# Autodesk Inventor assembly: claws_endeffector_4
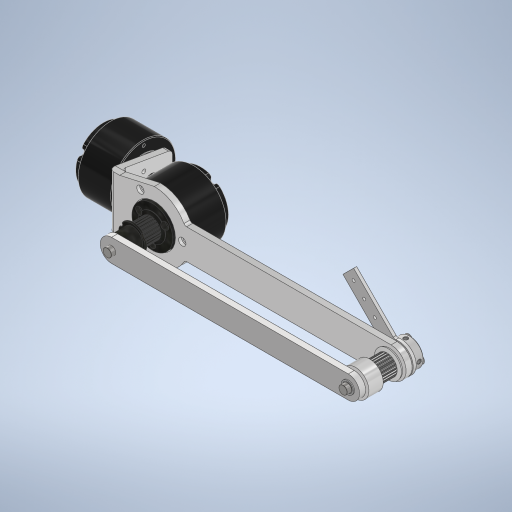
[picture p0: Inventor's stored thumbnail of the model, 512x512]
Saved by Autodesk Inventor 2024 (Build 280153000, 153)
## iProperties
Created: 2025-03-25
Part Number: claws_endeffector_4
Document SubType Name: Assembly
Designer: 1412z
Author: 1412z
## Documents named in this file (13)
- C:\Users\1412z\OneDrive\デスクトップ\rdclab\harvesting_robot\harvesting_endeffector\claws_endeffector\claws_endeffector_4.iam
- C:\Users\1412z\OneDrive\デスクトップ\rdclab\harvesting_robot\harvesting_endeffector\claws_endeffector\motor_holder\motor_holder_4.ipt
- C:\Users\1412z\OneDrive\デスクトップ\rdclab\harvesting_robot\harvesting_endeffector\claws_endeffector\GIM3505-08\GIM3505-8_with-driver.ipt
- C:\Users\1412z\OneDrive\デスクトップ\rdclab\harvesting_robot\harvesting_endeffector\claws_endeffector\misumi\SFL674ZZ_Autodesk_Inventor_2024_20250304\SFL674ZZ.ipt
- C:\Users\1412z\OneDrive\デスクトップ\rdclab\harvesting_robot\harvesting_endeffector\claws_endeffector\misumi\simring\simring_Φ4-Φ5.ipt
- C:\Users\1412z\OneDrive\デスクトップ\rdclab\harvesting_robot\harvesting_endeffector\claws_endeffector\misumi\HTPA22S2M100-K-P4_Autodesk_Inventor_2024_20250304\AIS2024\HTPA22S2M100-K-P4_a.ipt
- C:\Users\1412z\OneDrive\デスクトップ\rdclab\harvesting_robot\harvesting_endeffector\claws_endeffector\cutter_part\cutter_board.ipt
- C:\Users\1412z\OneDrive\デスクトップ\rdclab\harvesting_robot\harvesting_endeffector\claws_endeffector\misumi\SSCMN4_Autodesk_Inventor_2024_20250310\AIS2024\SSCMN4b.ipt
- C:\Users\1412z\OneDrive\デスクトップ\rdclab\harvesting_robot\harvesting_endeffector\claws_endeffector\misumi\M3×8\M3×8.ipt
- C:\Users\1412z\OneDrive\デスクトップ\rdclab\harvesting_robot\harvesting_endeffector\claws_endeffector\misumi\HTPA22S2M100-A-V4-Z6-J3_Autodesk_Inventor_2024_20250304\HTPA22S2M100-A-V4-Z6-J3_0_a-2.ipt
- C:\Users\1412z\OneDrive\デスクトップ\rdclab\harvesting_robot\harvesting_endeffector\claws_endeffector\motor_holder\motor_holder_top.ipt
- C:\Users\1412z\OneDrive\デスクトップ\rdclab\harvesting_robot\harvesting_endeffector\claws_endeffector\misumi\shaft\shaft_41.7mm.ipt
- C:\Users\1412z\OneDrive\デスクトップ\rdclab\harvesting_robot\harvesting_endeffector\claws_endeffector\misumi\shaft\shaft_24mm.ipt
## Components (26 placed, 12 different names)
1. motor_holder_4:1 — 回転:1, 回転:2, 回転:3, 回転:4, 回転:5, 回転:6
2. GIM3505-8_with-driver:1 — 回転:1, 回転:2, 回転:22, 回転:23
3. GIM3505-8_with-driver:2 — 回転:3, 回転:4
4. SFL674ZZ:1 — 回転:5, 回転:7
5. SFL674ZZ:2 — 回転:6, 回転:8
6. simring_Φ4-Φ5:1 — 回転:8, 回転:9
7. simring_Φ4-Φ5:2 — 回転:7, 回転:10
8. HTPA22S2M100-K-P4_a:1 — 回転:9, 回転:19
9. cutter_board:1 — 回転:10, 回転:11, 回転:12
10. SSCMN4b:1 — 回転:11, 回転:12, 回転:13, 回転:14, 回転:30
11. M3×8:1 — 回転:13
12. M3×8:2 — 回転:14
13. simring_Φ4-Φ5:4 — 回転:19, 回転:28
14. simring_Φ4-Φ5:5
15. HTPA22S2M100-A-V4-Z6-J3_0_a-2:1 — 回転:20, 回転:22, 回転:23, 回転:24
16. SFL674ZZ:3 — 回転:20, 回転:21
17. M3×8:3 — 回転:21
18. SFL674ZZ:4 — 回転:24, 回転:25
19. simring_Φ4-Φ5:6 — 回転:25, 回転:29
20. SFL674ZZ:5 — 回転:26, 回転:28
21. SFL674ZZ:6 — 回転:27
22. motor_holder_top:1 — 回転:26, 回転:27, 回転:29, 回転:32
23. shaft_41.7mm:1 — 回転:30, 回転:31
24. M3×8:4 — 回転:31
25. M3×8:5 — 回転:33
26. shaft_24mm:1 — 回転:32, 回転:33
## Relationships (29: RevoluteJoint 29)
- 回転:1 [RevoluteJoint]: motor_holder_4:1 ↔ GIM3505-8_with-driver:1
- 回転:2 [RevoluteJoint]: motor_holder_4:1 ↔ GIM3505-8_with-driver:1
- 回転:3 [RevoluteJoint]: motor_holder_4:1 ↔ GIM3505-8_with-driver:2
- 回転:4 [RevoluteJoint]: motor_holder_4:1 ↔ GIM3505-8_with-driver:2
- 回転:5 [RevoluteJoint]: motor_holder_4:1 ↔ SFL674ZZ:1
- 回転:6 [RevoluteJoint]: motor_holder_4:1 ↔ SFL674ZZ:2
- 回転:7 [RevoluteJoint]: SFL674ZZ:1 ↔ simring_Φ4-Φ5:2
- 回転:8 [RevoluteJoint]: SFL674ZZ:2 ↔ simring_Φ4-Φ5:1
- 回転:9 [RevoluteJoint]: simring_Φ4-Φ5:1 ↔ HTPA22S2M100-K-P4_a:1
- 回転:10 [RevoluteJoint]: simring_Φ4-Φ5:2 ↔ cutter_board:1
- 回転:11 [RevoluteJoint]: cutter_board:1 ↔ SSCMN4b:1
- 回転:12 [RevoluteJoint]: cutter_board:1 ↔ SSCMN4b:1
- 回転:13 [RevoluteJoint]: SSCMN4b:1 ↔ M3×8:1
- 回転:14 [RevoluteJoint]: SSCMN4b:1 ↔ M3×8:2
- 回転:19 [RevoluteJoint]: HTPA22S2M100-K-P4_a:1 ↔ simring_Φ4-Φ5:4
- 回転:20 [RevoluteJoint]: HTPA22S2M100-A-V4-Z6-J3_0_a-2:1 ↔ SFL674ZZ:3
- 回転:21 [RevoluteJoint]: SFL674ZZ:3 ↔ M3×8:3
- 回転:22 [RevoluteJoint]: GIM3505-8_with-driver:1 ↔ HTPA22S2M100-A-V4-Z6-J3_0_a-2:1
- 回転:23 [RevoluteJoint]: GIM3505-8_with-driver:1 ↔ HTPA22S2M100-A-V4-Z6-J3_0_a-2:1
- 回転:24 [RevoluteJoint]: HTPA22S2M100-A-V4-Z6-J3_0_a-2:1 ↔ SFL674ZZ:4
- 回転:25 [RevoluteJoint]: SFL674ZZ:4 ↔ simring_Φ4-Φ5:6
- 回転:26 [RevoluteJoint]: SFL674ZZ:5 ↔ motor_holder_top:1
- 回転:27 [RevoluteJoint]: SFL674ZZ:6 ↔ motor_holder_top:1
- 回転:28 [RevoluteJoint]: simring_Φ4-Φ5:4 ↔ SFL674ZZ:5
- 回転:29 [RevoluteJoint]: simring_Φ4-Φ5:6 ↔ motor_holder_top:1
- 回転:30 [RevoluteJoint]: SSCMN4b:1 ↔ shaft_41.7mm:1
- 回転:31 [RevoluteJoint]: shaft_41.7mm:1 ↔ M3×8:4
- 回転:32 [RevoluteJoint]: motor_holder_top:1 ↔ shaft_24mm:1
- 回転:33 [RevoluteJoint]: M3×8:5 ↔ shaft_24mm:1
